# Autodesk Inventor assembly: Assembly
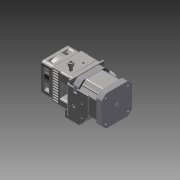
[picture p0: Inventor's stored thumbnail of the model, 180x180]
Saved by Autodesk Inventor 2017 (Build 210142000, 142)
## iProperties
Created: 2016-09-18
Part Number: Assembly
Document SubType Name: Assembly
Designer: user
Author: user
## Documents named in this file (7)
- C:\Projects\MK8Bracket\Inventor\Assembly.iam
- C:\Projects\MK8Bracket\Inventor\Bracket.ipt
- C:\Projects\MK8Bracket\Inventor\ExtruderParts\cog.ipt
- C:\Projects\MK8Bracket\Inventor\ExtruderParts\ExtruderPart.ipt
- C:\Projects\MK8Bracket\Inventor\ExtruderParts\StepperBack.ipt
- C:\Projects\MK8Bracket\Inventor\ExtruderParts\StepperBody.ipt
- C:\Projects\MK8Bracket\Inventor\ExtruderParts\StepperFront.ipt
## Components (6 placed, 6 different names)
1. Bracket:1 — Insert:2, Angle:1, Insert:3
2. cog:1 — Insert:6
3. ExtruderPart:1 — Insert:2, Angle:1, Insert:6
4. StepperBack:1 — Insert:5
5. StepperBody:1 — Insert:4, Insert:5
6. StepperFront:1 — Insert:3, Insert:4
## Relationships (6: Insert 5, Angle 1)
- Insert:2: Bracket:1 ↔ ExtruderPart:1
- Angle:1 (0 deg): Bracket:1 ↔ ExtruderPart:1
- Insert:3: Bracket:1 ↔ StepperFront:1
- Insert:4: StepperBody:1 ↔ StepperFront:1
- Insert:5: StepperBack:1 ↔ StepperBody:1
- Insert:6: cog:1 ↔ ExtruderPart:1
